# Autodesk Inventor assembly: HHSP25
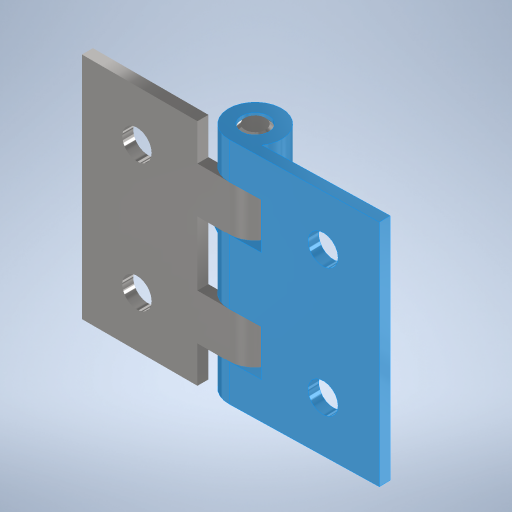
[picture p0: Inventor's stored thumbnail of the model, 512x512]
Saved by Autodesk Inventor 2023 (Build 270158000, 158)
## iProperties
Created: 2020-01-06
Part Number: HHSP25
Description: STEP AP203
Document SubType Name: Assembly
Designer: Hagihara Yuya
Sending System: PARTsolutions
Title: p:/temp/worker_6/temp/exporttempdir_3032_2252_TwEjh/format_0/HHSP25.stp
Revision Number: NONE
## Documents named in this file (4)
- C:\Users\kei\Desktop\新入生\BasicParts\Hinge\HHSP25\HHSP25.iam
- C:\Users\kei\Desktop\新入生\BasicParts\Hinge\HHSP25\_HHSP25-LEAF1.ipt
- C:\Users\kei\Desktop\新入生\BasicParts\Hinge\HHSP25\_HHSP25-LEAF2.ipt
- C:\Users\kei\Desktop\新入生\BasicParts\Hinge\HHSP25\_HHSP25-PIN.ipt
## Components (3 placed, 3 different names)
1. NAUO1 — 回転:1
2. NAUO2 — 回転:1, 回転:2
3. NAUO3 — 回転:2
## Relationships (2: RevoluteJoint 2)
- 回転:1 [RevoluteJoint]: NAUO1 ↔ NAUO2
- 回転:2 [RevoluteJoint]: NAUO2 ↔ NAUO3
